# Autodesk Inventor assembly: Sheet jukebox
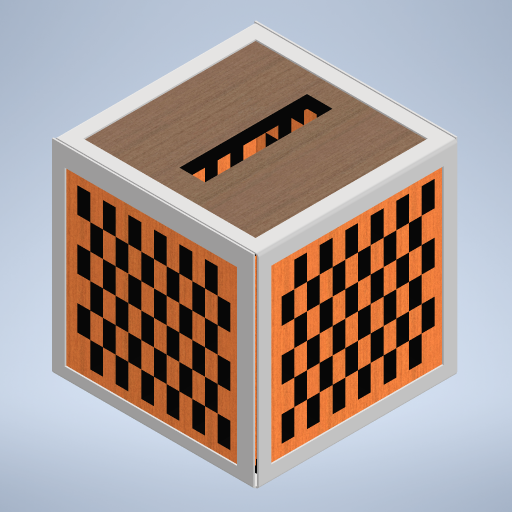
[picture p0: Inventor's stored thumbnail of the model, 512x512]
Saved by Autodesk Inventor 2024 (Build 280153000, 153)
## iProperties
Created: 2023-05-30
Part Number: Sheet jukebox
Document SubType Name: Assembly
Designer: newic
Author: newic
## Documents named in this file (5)
- D:\.My Models\.Inventor\Jukebox Project\Sheet jukebox.iam
- D:\.My Models\.Inventor\Jukebox Project\sheet metal frame.ipt
- D:\.My Models\.Inventor\Jukebox Project\JukeBox Outside panel sharp edges magnet slit.ipt
- D:\.My Models\.Inventor\Jukebox Project\JukeBox Bottem Panel.ipt
- D:\.My Models\.Inventor\Jukebox Project\JukeBox Top Panel SQ.ipt
## Components (7 placed, 4 different names)
1. sheet metal frame:1 — Mate:1, Mate:2, Mate:3, Mate:4, Mate:5, Mate:6, Mate:7, Mate:8, Mate:9, Mate:10, Mate:11, Mate:12, Mate:13, Mate:14, Mate:15, Mate:16, Mate:17, Mate:18
2. JukeBox Outside panel sharp edges magnet slit:1 — Mate:1, Mate:2, Mate:3
3. JukeBox Outside panel sharp edges magnet slit:2 — Mate:4, Mate:5, Mate:6
4. JukeBox Outside panel sharp edges magnet slit:3 — Mate:7, Mate:8, Mate:9
5. JukeBox Outside panel sharp edges magnet slit:4 — Mate:10, Mate:11, Mate:12
6. JukeBox Bottem Panel:1 — Mate:16, Mate:17, Mate:18
7. JukeBox Top Panel SQ:1 — Mate:13, Mate:14, Mate:15
## Relationships (18: Mate 18)
- Mate:1: sheet metal frame:1 ↔ JukeBox Outside panel sharp edges magnet slit:1
- Mate:2 (25.4 mm): sheet metal frame:1 ↔ JukeBox Outside panel sharp edges magnet slit:1
- Mate:3 (30.48 mm): sheet metal frame:1 ↔ JukeBox Outside panel sharp edges magnet slit:1
- Mate:4: sheet metal frame:1 ↔ JukeBox Outside panel sharp edges magnet slit:2
- Mate:5 (25.4 mm): sheet metal frame:1 ↔ JukeBox Outside panel sharp edges magnet slit:2
- Mate:6 (25.4 mm): sheet metal frame:1 ↔ JukeBox Outside panel sharp edges magnet slit:2
- Mate:7: sheet metal frame:1 ↔ JukeBox Outside panel sharp edges magnet slit:3
- Mate:8 (25.4 mm): sheet metal frame:1 ↔ JukeBox Outside panel sharp edges magnet slit:3
- Mate:9 (25.4 mm): sheet metal frame:1 ↔ JukeBox Outside panel sharp edges magnet slit:3
- Mate:10: sheet metal frame:1 ↔ JukeBox Outside panel sharp edges magnet slit:4
- Mate:11 (25.4 mm): sheet metal frame:1 ↔ JukeBox Outside panel sharp edges magnet slit:4
- Mate:12 (25.4 mm): sheet metal frame:1 ↔ JukeBox Outside panel sharp edges magnet slit:4
- Mate:13: sheet metal frame:1 ↔ JukeBox Top Panel SQ:1
- Mate:14 (25.4 mm): sheet metal frame:1 ↔ JukeBox Top Panel SQ:1
- Mate:15 (25.4 mm): sheet metal frame:1 ↔ JukeBox Top Panel SQ:1
- Mate:16: sheet metal frame:1 ↔ JukeBox Bottem Panel:1
- Mate:17 (25.4 mm): sheet metal frame:1 ↔ JukeBox Bottem Panel:1
- Mate:18 (25.4 mm): sheet metal frame:1 ↔ JukeBox Bottem Panel:1
